# Autodesk Inventor assembly: Complete Robot 1
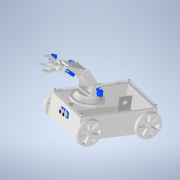
[picture p0: Inventor's stored thumbnail of the model, 180x180]
Saved by Autodesk Inventor 2022 (Build 260153000, 153)
## iProperties
Created: 2021-07-07
Part Number: Complete Robot 1
Document SubType Name: Assembly
Designer: USER
Author: USER
## Documents named in this file (5)
- F:\BVB\robotic arm\Complete Robot 1.iam
- F:\BVB\robotic arm\Completed Robot.iam
- F:\BVB\robotic arm\3rd arm motor pin.ipt
- F:\BVB\Switch 1\Pololu #1402 Snap-Action Switch.ipt
- F:\BVB\LED\Files\LED_Complete.iam
## Components (4 placed, 4 different names)
1. Completed Robot:1 [sub-assembly] — Mate:13, Flush:7, Mate:16, Flush:9, Flush:10, Mate:17, Flush:11, Flush:12
2. 3rd arm motor pin:1 — Mate:13, Flush:7
3. Pololu #1402 Snap-Action Switch:1 — Mate:16, Flush:9, Flush:10
4. LED_Complete:1 [sub-assembly] — Mate:17, Flush:11, Flush:12
## Relationships (8: Flush 5, Mate 3)
- Mate:13: Completed Robot:1 ↔ 3rd arm motor pin:1
- Flush:7: Completed Robot:1 ↔ 3rd arm motor pin:1
- Mate:16 (-9 mm): Completed Robot:1 ↔ Pololu #1402 Snap-Action Switch:1
- Flush:9 (-60 mm): Completed Robot:1 ↔ Pololu #1402 Snap-Action Switch:1
- Flush:10 (-40 mm): Completed Robot:1 ↔ Pololu #1402 Snap-Action Switch:1
- Mate:17 (-2 mm): Completed Robot:1 ↔ LED_Complete:1
- Flush:11 (30 mm): Completed Robot:1 ↔ LED_Complete:1
- Flush:12 (-50 mm): Completed Robot:1 ↔ LED_Complete:1
